# Autodesk Inventor assembly: All_Part
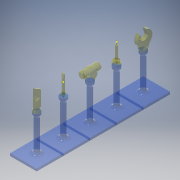
[picture p0: Inventor's stored thumbnail of the model, 180x180]
Saved by Autodesk Inventor 2017 (Build 210142000, 142)
## iProperties
Created: 2021-02-25
Part Number: All_Part
Document SubType Name: Assembly
Designer: Lenovo Y900
Author: Lenovo Y900
## Documents named in this file (6)
- D:\Sekolah\Skripsi\New Part\All_Part.iam
- D:\Sekolah\Skripsi\New Part\Assembly_Cutter.iam
- D:\Sekolah\Skripsi\New Part\Assembly_Obeng.iam
- D:\Sekolah\Skripsi\New Part\Assembly_Palu.iam
- D:\Sekolah\Skripsi\New Part\Assembly_Solder.iam
- D:\Sekolah\Skripsi\New Part\Assembly_Spanner.iam
## Components (5 placed, 5 different names)
1. Assembly_Cutter:1 [sub-assembly] — Flush:1, Flush:5
2. Assembly_Obeng:1 [sub-assembly] — Flush:1, Flush:2, Flush:5, Flush:6
3. Assembly_Palu:1 [sub-assembly] — Flush:2, Flush:3, Flush:6, Flush:7
4. Assembly_Solder:1 [sub-assembly] — Flush:3, Flush:4, Flush:7, Flush:8
5. Assembly_Spanner:1 [sub-assembly] — Flush:4, Flush:8
## Relationships (8: Flush 8)
- Flush:1: Assembly_Cutter:1 ↔ Assembly_Obeng:1
- Flush:2: Assembly_Obeng:1 ↔ Assembly_Palu:1
- Flush:3: Assembly_Palu:1 ↔ Assembly_Solder:1
- Flush:4: Assembly_Solder:1 ↔ Assembly_Spanner:1
- Flush:5: Assembly_Cutter:1 ↔ Assembly_Obeng:1
- Flush:6: Assembly_Obeng:1 ↔ Assembly_Palu:1
- Flush:7: Assembly_Palu:1 ↔ Assembly_Solder:1
- Flush:8: Assembly_Solder:1 ↔ Assembly_Spanner:1
